# Autodesk Inventor assembly: worm gearbox nmrv 40
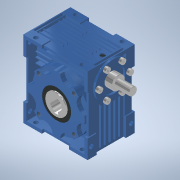
[picture p0: Inventor's stored thumbnail of the model, 180x180]
Saved by Autodesk Inventor 2020 (Build 240168000, 168)
## iProperties
Created: 2020-08-01
Part Number: worm gearbox nmrv 40
Document SubType Name: Assembly
Designer: Vikki
Author: Vikki
## Documents named in this file (4)
- E:\project inventor pro\flipkart grid models\articulated arm\worm gearbox nmrv 40.iam
- E:\project inventor pro\flipkart grid models\articulated arm\nmrv 40 30 to1 casing.ipt
- E:\project inventor pro\flipkart grid models\articulated arm\input shaft nmrv-40.ipt
- E:\project inventor pro\flipkart grid models\articulated arm\outputshaft nmrv-40.ipt
## Components (3 placed, 3 different names)
1. nmrv 40 30 to1 casing:1 — Mate:1, Mate:2, Mate:3, Flush:1
2. input shaft nmrv-40:1 — Mate:1, Mate:2, Rotation:1
3. outputshaft nmrv-40:1 — Mate:3, Flush:1, Rotation:1
## Relationships (5: Mate 3, Flush 1, RelateRotation 1)
- Mate:1: nmrv 40 30 to1 casing:1 ↔ input shaft nmrv-40:1
- Mate:2: nmrv 40 30 to1 casing:1 ↔ input shaft nmrv-40:1
- Mate:3: nmrv 40 30 to1 casing:1 ↔ outputshaft nmrv-40:1
- Flush:1 (-1 mm): nmrv 40 30 to1 casing:1 ↔ outputshaft nmrv-40:1
- Rotation:1 [RelateRotation] (30 ul): input shaft nmrv-40:1 ↔ outputshaft nmrv-40:1
